# Autodesk Inventor assembly: POS 12
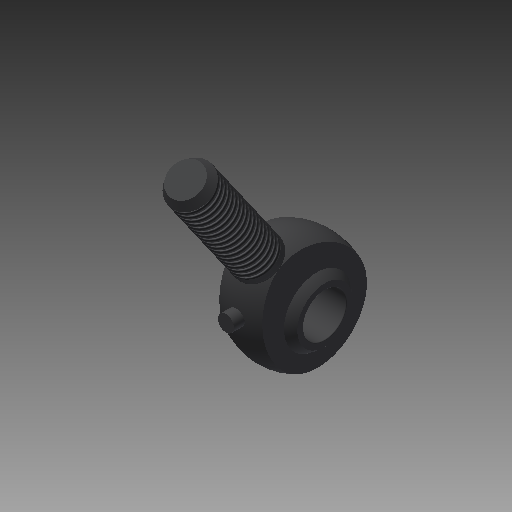
[picture p0: Inventor's stored thumbnail of the model, 512x512]
Saved by Autodesk Inventor 2018 (Build 220112000, 112)
## iProperties
Category: PARTsolutions
Company: IKO
Created: 2017-09-12
Part Number: POS 12
Catalog Web Link: www.cadenas.de
Description: Rod-End-with Male Thread (POS)-
Vendor: IKO
Document SubType Name: Assembly
Designer: psAdmin
Manufacturer: IKO
PSOL_IDENT_0: {$CADENAS_DATA\23d-libs\iko\iko_bearings\pillobals\insert_type\rod_end_with_mt_asmtab.prj},183 {VTYP=
PSOL_IDENT_1: 3D},{STYP=ASSTAB},{NB=POS 12},{LINA=POS 12},{NN=Rod-End-with Male Thread (POS)},{DATE=13.10.2016 10:
PSOL_IDENT_2: 02:13},{GEOMDATE=04.12.2007},{VERSION=},{LINEID=70},{LINESUBID=-1},{WBVAR=}  {NB=POS 12},{LINA=POS 1
PSOL_IDENT_3: 2},{KT=DUMMY},{IDNR=},{RID=G_70},{STDRT=12},{DESC=(gevmsg IKOSTV 914)},{TRNUMBER=},{PAST=A},{REST=O}
PSOL_IDENT_4: ,{ORDER=POS 12},{MASS=85.0},{SD=12},{G=M12x1.75},{NDM=12.000},{P1=1.750},{SD2=30},{C1=12.0},{B=16},{
PSOL_IDENT_5: SD1=15.4},{SL2=69},{SH=54},{SL1=33},{SR1=0.2},{DBL=22.23},{C2=0.00},{C3=0.00},{AA=0.00},{BB=0},{R2=3
PSOL_IDENT_6: .0},{R3=22.5},{H2=41.03},{CGN=4.5},{P=2.5},{C=60},{LL6=34.56},{LL7=0.00},{LL8=2.34},{LL9=0.00},{LL10=
PSOL_IDENT_7: 0.00},{SDK=22.225},{CD=13100},{CS=16900},{G1=12},{GG1=10.11},{PP=1.8},{ALFA=55},{BL=4},{SC=1},{PPATH=
PSOL_IDENT_8: rod_end_with_mt_asmtpl.prj}
NN: Rod-End-with Male Thread (POS)
NB: POS 12
NBSYN: $ORDER.
LINA: POS 12
ORDER: POS 12
MASS: 85.0
SD: 12
G: M12x1.75
SD2: 30
C1: 12.0
B: 16
SD1: 15.4
SL2: 69
SH: 54
SL1: 33
SR1: 0.2
SDK: 22.225
CD: 13100
CS: 16900
SUPPLIER: IKO
ARTICLENO: POS 12
BOMINFO: POS 12
CREATOR: CADENAS GmbH
Title: POS 12
Author: Cadenas PARTsolutions
## Documents named in this file (3)
- D:\Works\RBBR\CAD\汎用部品\ピロボール12mm\POS 12.iam
- D:\Works\RBBR\CAD\汎用部品\ピロボール12mm\POS 12 Body.ipt
- D:\Works\RBBR\CAD\汎用部品\ピロボール12mm\POS 12 Ball.ipt
## Components (2 placed, 2 different names)
1. POS 12 Body:1 — ボール:1
2. POS 12 Ball:1 — ボール:1
## Relationships (1: BallJoint 1)
- ボール:1 [BallJoint]: POS 12 Body:1 ↔ POS 12 Ball:1
